# Autodesk Inventor assembly: Auspressrolle_befaesstigung
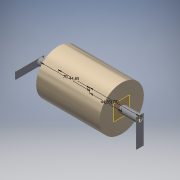
[picture p0: Inventor's stored thumbnail of the model, 180x180]
Saved by Autodesk Inventor 2018 (Build 220112000, 112)
## iProperties
Created: 2018-01-12
Part Number: Auspressrolle_befaesstigung
Material: Generisch
Document SubType Name: Assembly
Designer: Julian
Author: Julian
## Documents named in this file (4)
- C:\Users\Julian\Desktop\Schule\5AHME\Diplomarbeit\Git\fuettr_prototype\Mechanical\Inventorskizzen\Auspressrolle_befaesstigung.iam
- C:\Users\Julian\Desktop\Schule\5AHME\Diplomarbeit\Git\fuettr_prototype\Mechanical\Inventorskizzen\Auspressrolle.ipt
- C:\Users\Julian\Desktop\Schule\5AHME\Diplomarbeit\Git\fuettr_prototype\Mechanical\Inventorskizzen\Verbindungsstück_Rolle.ipt
- C:\Users\Julian\Desktop\Schule\5AHME\Diplomarbeit\Git\fuettr_prototype\Mechanical\Inventorskizzen\Kunststoffrolle_antrieb.ipt
## Components (4 placed, 3 different names)
1. Auspressrolle:1 — Starr:1, Starr:2, Passend:1, Fluchtend:1
2. Verbindungsstück_Rolle:1 — Starr:1
3. Verbindungsstück_Rolle:2 — Starr:2
4. Kunststoffrolle_antrieb:1 — Passend:1, Fluchtend:1
## Relationships (4: WeldJoint 2, Mate 1, Flush 1)
- Starr:1 [WeldJoint]: Auspressrolle:1 ↔ Verbindungsstück_Rolle:1
- Starr:2 [WeldJoint]: Auspressrolle:1 ↔ Verbindungsstück_Rolle:2
- Passend:1 [Mate]: Auspressrolle:1 ↔ Kunststoffrolle_antrieb:1
- Fluchtend:1 [Flush]: Auspressrolle:1 ↔ Kunststoffrolle_antrieb:1
